# Autodesk Inventor assembly: assembly
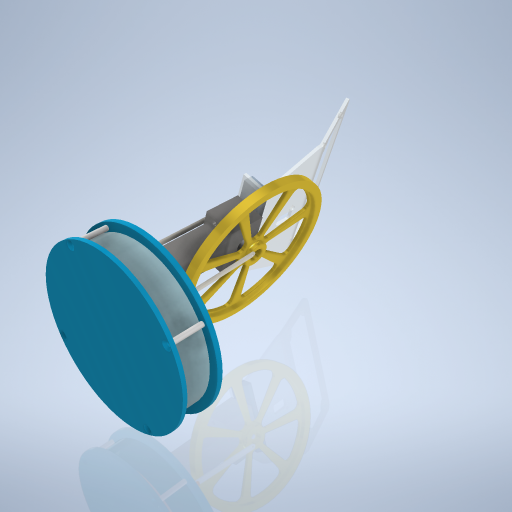
[picture p0: Inventor's stored thumbnail of the model, 512x512]
Saved by Autodesk Inventor 2024.2 (Build 282272000, 272)
## iProperties
Created: 2024-04-06
Part Number: assembly
Document SubType Name: Assembly
Designer: Fabri
Author: Fabri
## Documents named in this file (19)
- C:\Users\Fabri\Documents\Inventor\Stirlingmotor\assembly.iam
- C:\Users\Fabri\Documents\Inventor\Stirlingmotor\plate.ipt
- C:\Users\Fabri\Documents\Inventor\Stirlingmotor\cylinder.ipt
- C:\Users\Fabri\Documents\Inventor\Stirlingmotor\steuerkolben.ipt
- C:\Users\Fabri\Documents\Inventor\Stirlingmotor\stange.ipt
- C:\Users\Fabri\Documents\Inventor\Stirlingmotor\plate_2.ipt
- C:\Users\Fabri\Documents\Inventor\Stirlingmotor\Lagerbock.ipt
- C:\Users\Fabri\Documents\Inventor\Stirlingmotor\Ak zylinder.ipt
- C:\Users\Fabri\Documents\Inventor\Stirlingmotor\Arbeitskolben.ipt
- C:\Users\Fabri\Documents\Inventor\Stirlingmotor\Gewindehülse.ipt
- C:\Users\Fabri\Documents\Inventor\Stirlingmotor\Führungsbüchse.ipt
- C:\Users\Fabri\Documents\Inventor\Stirlingmotor\kopf.ipt
- C:\Users\Fabri\Documents\Inventor\Stirlingmotor\pleuelstange.ipt
- C:\Users\Fabri\Documents\Inventor\Stirlingmotor\Rad.ipt
- C:\Users\Fabri\Documents\Inventor\Stirlingmotor\Kurbel.ipt
- C:\Users\Fabri\Documents\Inventor\Stirlingmotor\Glaswinkel.ipt
- C:\Users\Fabri\Documents\Inventor\Stirlingmotor\Flach_Alu.ipt
- C:\Users\Fabri\Documents\Inventor\Stirlingmotor\büchse.ipt
- C:\Users\Fabri\Documents\Inventor\Stirlingmotor\kurbelwelle.ipt
## Components (24 placed, 18 different names)
1. plate:1 — Einfügen:1, Einfügen:2, Passend:1
2. cylinder:1 — Einfügen:1
3. steuerkolben:1 — Einfügen:2, Einfügen:3
4. stange:1 — Einfügen:3, Einfügen:4, Einfügen:12, Passend:4
5. plate_2:1 — Einfügen:4, Einfügen:5, Winkel:1, Einfügen:6, Einfügen:8, Einfügen:9, Einfügen:10, Einfügen:11
6. Lagerbock:1 — Einfügen:5, Winkel:1, Winkel:2, Winkel:3, Einfügen:17, Winkel:4, Einfügen:18, Fluchtend:1, Einfügen:20, Passend:6
7. Ak zylinder:1 — Einfügen:6, Einfügen:7
8. Arbeitskolben:1 — Einfügen:7, Einfügen:14
9. Gewindehülse:1 — Einfügen:11
10. Gewindehülse:2 — Einfügen:8, Passend:2, Passend:3
11. Gewindehülse:3 — Einfügen:9
12. Gewindehülse:4 — Einfügen:10
13. Führungsbüchse:1 — Einfügen:12
14. kopf:1 — Passend:4, Winkel:2, Einfügen:13
15. pleuelstange:1 — Einfügen:13
16. Rad:1 — Passend:5, Einfügen:21
17. stange:2 — Einfügen:14, Einfügen:15
18. kopf:2 — Einfügen:15, Winkel:3, Einfügen:16
19. pleuelstange:2 — Einfügen:16
20. Kurbel:1 — Einfügen:17, Winkel:4
21. Glaswinkel:1 — Einfügen:18, Fluchtend:1, Einfügen:19, Fluchtend:2
22. Flach_Alu:1 — Einfügen:19, Fluchtend:2
23. büchse:1 — Einfügen:20
24. kurbelwelle:1 — Einfügen:21
## Relationships (34: Insert 21, Mate 7, Angle 4, Flush 2)
- Einfügen:1 [Insert]: plate:1 ↔ cylinder:1
- Einfügen:2 [Insert]: plate:1 ↔ steuerkolben:1
- Einfügen:3 [Insert] (-7 mm): steuerkolben:1 ↔ stange:1
- Einfügen:4 [Insert] (-17.5 mm): stange:1 ↔ plate_2:1
- Einfügen:5 [Insert]: plate_2:1 ↔ Lagerbock:1
- Winkel:1 [Angle] (180 deg): plate_2:1 ↔ Lagerbock:1
- Einfügen:6 [Insert]: plate_2:1 ↔ Ak zylinder:1
- Einfügen:7 [Insert] (-15 mm): Ak zylinder:1 ↔ Arbeitskolben:1
- Einfügen:8 [Insert] (-19 mm): plate_2:1 ↔ Gewindehülse:2
- Passend:1 [Mate]: plate:1
- Passend:2 [Mate]: Gewindehülse:2
- Passend:3 [Mate]: Gewindehülse:2
- Einfügen:9 [Insert] (-21 mm): plate_2:1 ↔ Gewindehülse:3
- Einfügen:10 [Insert] (-21 mm): plate_2:1 ↔ Gewindehülse:4
- Einfügen:11 [Insert] (-21 mm): plate_2:1 ↔ Gewindehülse:1
- Einfügen:12 [Insert] (-13.5 mm): stange:1 ↔ Führungsbüchse:1
- Passend:4 [Mate]: stange:1 ↔ kopf:1
- Winkel:2 [Angle] (0 deg): Lagerbock:1 ↔ kopf:1
- Einfügen:13 [Insert] (0.1 mm): kopf:1 ↔ pleuelstange:1
- Einfügen:14 [Insert] (-25.2 mm): Arbeitskolben:1 ↔ stange:2
- Einfügen:15 [Insert] (-2 mm): stange:2 ↔ kopf:2
- Winkel:3 [Angle] (0 deg): Lagerbock:1 ↔ kopf:2
- Einfügen:16 [Insert]: kopf:2 ↔ pleuelstange:2
- Einfügen:17 [Insert] (-0.9 mm): Lagerbock:1 ↔ Kurbel:1
- Winkel:4 [Angle] (90 deg): Lagerbock:1 ↔ Kurbel:1
- Einfügen:18 [Insert]: Lagerbock:1 ↔ Glaswinkel:1
- Fluchtend:1 [Flush]: Lagerbock:1 ↔ Glaswinkel:1
- Einfügen:19 [Insert]: Glaswinkel:1 ↔ Flach_Alu:1
- Fluchtend:2 [Flush]: Glaswinkel:1 ↔ Flach_Alu:1
- Einfügen:20 [Insert] (-15 mm): Lagerbock:1 ↔ büchse:1
- Passend:5 [Mate]: Rad:1
- Passend:6 [Mate]: Lagerbock:1
- Passend:7 [Mate]
- Einfügen:21 [Insert] (-25 mm): Rad:1 ↔ kurbelwelle:1
